# Autodesk Inventor assembly: InternalElectronics
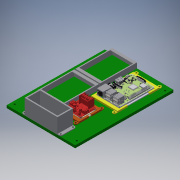
[picture p0: Inventor's stored thumbnail of the model, 180x180]
Saved by Autodesk Inventor 2018 (Build 220112000, 112)
## iProperties
Created: 2018-07-29
Part Number: InternalElectronics
Document SubType Name: Assembly
Designer: jklei
Author: jklei
## Documents named in this file (10)
- C:\Users\jklei\Desktop\Projects\Shamrock\Hardware\Electronics\InternalElectronics.iam
- C:\Users\jklei\Desktop\Projects\Shamrock\Hardware\Electronics\raspberry-pi\raspberry_pi_3_b_plus.iam
- C:\Users\jklei\Desktop\Projects\Shamrock\Hardware\Electronics\L298N.ipt
- C:\Users\jklei\Desktop\Projects\Shamrock\Hardware\Electronics\pi-holder.ipt
- C:\Users\jklei\Desktop\Projects\Shamrock\Hardware\Electronics\ModBoard-Bottom.ipt
- C:\Users\jklei\Desktop\Projects\Shamrock\Hardware\Electronics\Electronics-Wedge.ipt
- C:\Users\jklei\Desktop\Projects\Shamrock\Hardware\Electronics\L298N-holder.ipt
- C:\Users\jklei\Desktop\Projects\Shamrock\Hardware\Electronics\Electronics-Wedge-small.ipt
- C:\Users\jklei\Desktop\Projects\Shamrock\Hardware\Electronics\MiniBreadboardHolder.ipt
- C:\Users\jklei\Desktop\Projects\Shamrock\Hardware\Electronics\BatteryHolder.ipt
## Components (12 placed, 9 different names)
1. raspberry_pi_3_b_plus:1 [sub-assembly] — Insert:1, Insert:2
2. L298N:1 — Insert:14, Angle:4
3. pi-holder:1 — Insert:1, Insert:2, Mate:21, Mate:22, Mate:23, Mate:24, Mate:25
4. ModBoard-Bottom:1 — Insert:4, Insert:5, Mate:14, Insert:15, Angle:5, Angle:6, Insert:16, Insert:17, Angle:7, Insert:18
5. Electronics-Wedge:2 — Mate:24, Mate:25, Flush:3
6. Electronics-Wedge:3 — Insert:4, Insert:5, Mate:21, Mate:22, Mate:23, Flush:3
7. L298N-holder:1 — Insert:14, Angle:4, Mate:15, Mate:16, Mate:17, Mate:18, Mate:19, Mate:20
8. Electronics-Wedge-small:1 — Mate:14, Mate:15, Mate:16, Mate:17, Insert:15
9. Electronics-Wedge-small:2 — Mate:18, Mate:19, Mate:20, Angle:5
10. MiniBreadboardHolder:1 — Angle:6, Insert:16
11. MiniBreadboardHolder:2 — Insert:17, Angle:7
12. BatteryHolder:1 — Insert:18
## Relationships (26: Mate 12, Insert 9, Angle 4, Flush 1)
- Insert:1: raspberry_pi_3_b_plus:1 ↔ pi-holder:1
- Insert:2: raspberry_pi_3_b_plus:1 ↔ pi-holder:1
- Insert:4: ModBoard-Bottom:1 ↔ Electronics-Wedge:3
- Insert:5: ModBoard-Bottom:1 ↔ Electronics-Wedge:3
- Insert:14: L298N:1 ↔ L298N-holder:1
- Angle:4 (0 deg): L298N:1 ↔ L298N-holder:1
- Mate:14: ModBoard-Bottom:1 ↔ Electronics-Wedge-small:1
- Mate:15: L298N-holder:1 ↔ Electronics-Wedge-small:1
- Mate:16: L298N-holder:1 ↔ Electronics-Wedge-small:1
- Mate:17: L298N-holder:1 ↔ Electronics-Wedge-small:1
- Mate:18: L298N-holder:1 ↔ Electronics-Wedge-small:2
- Mate:19: L298N-holder:1 ↔ Electronics-Wedge-small:2
- Mate:20: L298N-holder:1 ↔ Electronics-Wedge-small:2
- Mate:21: pi-holder:1 ↔ Electronics-Wedge:3
- Mate:22: pi-holder:1 ↔ Electronics-Wedge:3
- Mate:23: pi-holder:1 ↔ Electronics-Wedge:3
- Mate:24: pi-holder:1 ↔ Electronics-Wedge:2
- Mate:25: pi-holder:1 ↔ Electronics-Wedge:2
- Flush:3: Electronics-Wedge:2 ↔ Electronics-Wedge:3
- Insert:15: ModBoard-Bottom:1 ↔ Electronics-Wedge-small:1
- Angle:5 (90 deg): ModBoard-Bottom:1 ↔ Electronics-Wedge-small:2
- Angle:6 (0 deg): ModBoard-Bottom:1 ↔ MiniBreadboardHolder:1
- Insert:16: ModBoard-Bottom:1 ↔ MiniBreadboardHolder:1
- Insert:17: ModBoard-Bottom:1 ↔ MiniBreadboardHolder:2
- Angle:7 (0 deg): ModBoard-Bottom:1 ↔ MiniBreadboardHolder:2
- Insert:18: ModBoard-Bottom:1 ↔ BatteryHolder:1
